# Autodesk Inventor assembly: Lamp
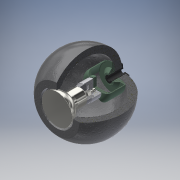
[picture p0: Inventor's stored thumbnail of the model, 180x180]
Saved by Autodesk Inventor 2018.2 (Build 222227000, 227)
## iProperties
Created: 2018-01-26
Part Number: Lamp
Material: Generisch
Document SubType Name: Assembly
Designer: JochenAlt
Author: JochenAlt
## Documents named in this file (6)
- D:\Projects\concretelamp\CAD\Lamp.iam
- D:\Projects\concretelamp\CAD\CableStrainRelief.ipt
- D:\Projects\concretelamp\CAD\Inlet.ipt
- D:\Projects\concretelamp\CAD\Lamp.ipt
- D:\Projects\concretelamp\CAD\Bulb GU10\Bulb GU10.iam
- D:\Projects\concretelamp\CAD\GU10-Socket.ipt
## Components (5 placed, 5 different names)
1. Kabelzugentlastung:1 — Passend:3, Passend:21, Passend:22, Passend:23
2. V5 Inlet:1 — Passend:22, Passend:23, Passend:24, Passend:25, Passend:26
3. Lamp:1 — Passend:3, Passend:21
4. Bulb GU10:1 [sub-assembly] — Passend:19, Passend:24, Passend:27, Passend:28
5. GU10-Socket:1 — Passend:19, Passend:25, Passend:26, Passend:27, Passend:28
## Relationships (10: Mate 10)
- Passend:3 [Mate]: Kabelzugentlastung:1 ↔ Lamp:1
- Passend:19 [Mate]: Bulb GU10:1 ↔ GU10-Socket:1
- Passend:21 [Mate]: Kabelzugentlastung:1 ↔ Lamp:1
- Passend:22 [Mate]: Kabelzugentlastung:1 ↔ V5 Inlet:1
- Passend:23 [Mate] (-2.8 mm): Kabelzugentlastung:1 ↔ V5 Inlet:1
- Passend:24 [Mate]: V5 Inlet:1 ↔ Bulb GU10:1
- Passend:25 [Mate]: V5 Inlet:1 ↔ GU10-Socket:1
- Passend:26 [Mate] (0.3 mm): V5 Inlet:1 ↔ GU10-Socket:1
- Passend:27 [Mate]: Bulb GU10:1 ↔ GU10-Socket:1
- Passend:28 [Mate] (0.3 mm): Bulb GU10:1 ↔ GU10-Socket:1
